# Autodesk Inventor assembly: wobble arm
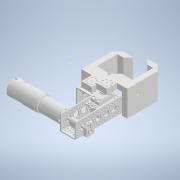
[picture p0: Inventor's stored thumbnail of the model, 180x180]
Saved by Autodesk Inventor 2020 (Build 240168000, 168)
## iProperties
Created: 2020-09-23
Part Number: wobble arm
Document SubType Name: Assembly
Designer: elois
Author: elois
## Documents named in this file (10)
- C:\Users\tdmp4\Documents\GitHub\CAD-2021-Ultimate_Goal\Wobble Goal\wobble arm.iam
- C:\Users\tdmp4\Documents\GitHub\CAD-2021-Ultimate_Goal\Wobble Goal\assembled servo block.iam
- C:\Users\tdmp4\Documents\GitHub\CAD-2021-Ultimate_Goal\Wobble Goal\wobble goal arm.ipt
- C:\Users\tdmp4\Documents\GitHub\CAD-2021-Ultimate_Goal\ServoCity\625051 assembly.ipt
- C:\Users\tdmp4\Documents\GitHub\CAD-2021-Ultimate_Goal\ServoCity\545588 assembly.ipt
- C:\Users\tdmp4\Documents\GitHub\CAD-2021-Ultimate_Goal\ServoCity\634158.ipt
- C:\Users\tdmp4\Documents\GitHub\CAD-2021-Ultimate_Goal\Wobble Goal\wobble goal arm_MIR1.ipt
- C:\Users\tdmp4\Documents\GitHub\CAD-2021-Ultimate_Goal\ServoCity\4 inch channel.ipt
- C:\Users\tdmp4\Documents\GitHub\CAD-2021-Ultimate_Goal\ServoCity\motor 188-1.ipt
- C:\Users\tdmp4\Documents\GitHub\CAD-2021-Ultimate_Goal\ServoCity\585440.ipt
## Components (9 placed, 9 different names)
1. assembled servo block:1 [sub-assembly] — Mate:2, Mate:3, Mate:7
2. 4 inch channel:1 — Mate:1, Mate:2, Mate:3, Mate:4, Mate:8
3. motor 188-1:1 — Mate:1, Mate:4, Mate:10, Mate:11
4. wobble goal arm:1 — Mate:7
5. 585440:1 — Mate:8, Mate:16, Mate:17
6. 625051 assembly:1 — Mate:10, Mate:11, Mate:12, Mate:13
7. 545588 assembly:1 — Mate:14, Mate:15
8. 634158:1 — Mate:12, Mate:13, Mate:14, Mate:15
9. wobble goal arm_MIR1:1 — Mate:16, Mate:17
## Relationships (14: Mate 14)
- Mate:1: 4 inch channel:1 ↔ motor 188-1:1
- Mate:2: assembled servo block:1 ↔ 4 inch channel:1
- Mate:3: assembled servo block:1 ↔ 4 inch channel:1
- Mate:4: 4 inch channel:1 ↔ motor 188-1:1
- Mate:7: assembled servo block:1 ↔ wobble goal arm:1
- Mate:8: 4 inch channel:1 ↔ 585440:1
- Mate:10: motor 188-1:1 ↔ 625051 assembly:1
- Mate:11: motor 188-1:1 ↔ 625051 assembly:1
- Mate:12: 625051 assembly:1 ↔ 634158:1
- Mate:13: 625051 assembly:1 ↔ 634158:1
- Mate:14: 545588 assembly:1 ↔ 634158:1
- Mate:15: 545588 assembly:1 ↔ 634158:1
- Mate:16: 585440:1 ↔ wobble goal arm_MIR1:1
- Mate:17: 585440:1 ↔ wobble goal arm_MIR1:1
